# Autodesk Inventor assembly: Assy_linear_module
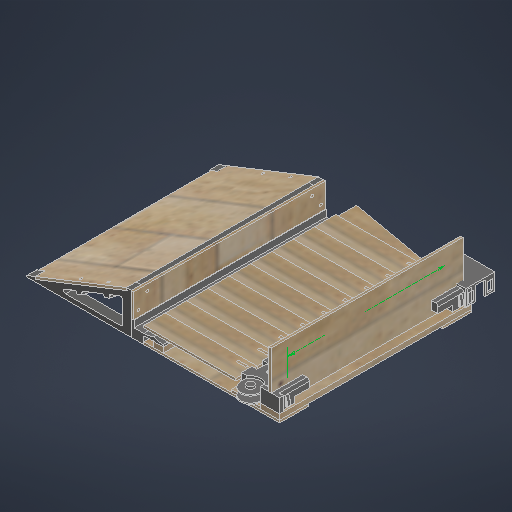
[picture p0: Inventor's stored thumbnail of the model, 512x512]
Saved by Autodesk Inventor 2026.3 (Build 303398000, 398)
## iProperties
Created: 2025-09-27
Part Number: Assy_linear_module
Document SubType Name: Assembly
Designer: hibik
Author: hibik
## Documents named in this file (15)
- D:\model\D2_Conveyor_2026\liniar_module\Assy_linear_module.iam
- D:\model\D2_Conveyor_2026\liniar_module\base.ipt
- D:\model\D2_Conveyor_2026\liniar_module\connector_base.ipt
- D:\model\D2_Conveyor_2026\liniar_module\back_upper.ipt
- D:\model\D2_Conveyor_2026\connectors\connector_male.ipt
- D:\model\D2_Conveyor_2026\liniar_module\belt_rail.ipt
- D:\model\D2_Conveyor_2026\liniar_module\front.ipt
- D:\model\D2_Conveyor_2026\belt\belt_linear.iam
- D:\model\D2_Conveyor_2026\liniar_module\front_rail.ipt
- D:\model\D2_Conveyor_2026\connectors\connetcor_female_cover.ipt
- D:\model\D2_Conveyor_2026\liniar_module\wall.ipt
- D:\model\D2_Conveyor_2026\liniar_module\Slope_Riner.ipt
- D:\model\D2_Conveyor_2026\liniar_module\Side_Wall_Riner.ipt
- D:\model\D2_Conveyor_2026\liniar_module\Spcer_Upper.ipt
- D:\model\D2_Conveyor_2026\liniar_module\Wall_Stand.ipt
## Components (17 placed, 14 different names)
1. base:1 — メイト:1, フラッシュ:1, フラッシュ:3, メイト:7, フラッシュ:7, フラッシュ:8, フラッシュ:9, メイト:12, フラッシュ:11
2. connector_base:1 — メイト:1, フラッシュ:1, フラッシュ:3, メイト:3, フラッシュ:5, フラッシュ:6, メイト:4, メイト:5, メイト:6, メイト:8, メイト:9, メイト:10, メイト:11, メイト:13, メイト:14, メイト:19
3. base:2 — メイト:3, フラッシュ:5, フラッシュ:6
4. connector_male:7 — メイト:9, メイト:10, メイト:11, メイト:16
5. connector_male:8 — メイト:4, メイト:5, メイト:6, メイト:17, メイト:18
6. belt_rail:1 — メイト:7, フラッシュ:7, メイト:8, 正接:1
7. front:1 — フラッシュ:8, フラッシュ:9, メイト:12, フラッシュ:12, フラッシュ:13, フラッシュ:14
8. back_upper:1 — フラッシュ:10, メイト:13, メイト:14, メイト:15
9. belt_linear:1 [sub-assembly] — メイト:15, 正接:1, フラッシュ:11
10. front_rail:1 — フラッシュ:12, フラッシュ:13, フラッシュ:14, フラッシュ:25, フラッシュ:26, メイト:24
11. connetcor_female_cover:1 — メイト:16
12. wall:1 — メイト:17, メイト:18, メイト:19
13. Slope_Riner:1 — メイト:20, メイト:21, フラッシュ:23, フラッシュ:24, メイト:22, メイト:23
14. Wall_Stand:2 — メイト:21, フラッシュ:23, メイト:23, フラッシュ:25, フラッシュ:26, メイト:24, 回転:1
15. Wall_Stand:3 — メイト:20, フラッシュ:24, メイト:22, メイト:25
16. Side_Wall_Riner:1 — メイト:25, 回転:1, メイト:26, 回転:2
17. Spcer_Upper:1 — メイト:26, 回転:2
## Relationships (44: Mate 25, Flush 16, RevoluteJoint 2, Tangent 1)
- メイト:1 [Mate]: base:1 ↔ connector_base:1
- フラッシュ:1 [Flush]: base:1 ↔ connector_base:1
- フラッシュ:3 [Flush]: base:1 ↔ connector_base:1
- メイト:3 [Mate]: connector_base:1 ↔ base:2
- フラッシュ:5 [Flush]: connector_base:1 ↔ base:2
- フラッシュ:6 [Flush]: connector_base:1 ↔ base:2
- メイト:4 [Mate]: connector_base:1 ↔ connector_male:8
- メイト:5 [Mate]: connector_base:1 ↔ connector_male:8
- メイト:6 [Mate]: connector_base:1 ↔ connector_male:8
- メイト:7 [Mate]: base:1 ↔ belt_rail:1
- フラッシュ:7 [Flush]: base:1 ↔ belt_rail:1
- メイト:8 [Mate]: connector_base:1 ↔ belt_rail:1
- メイト:9 [Mate]: connector_base:1 ↔ connector_male:7
- メイト:10 [Mate]: connector_base:1 ↔ connector_male:7
- メイト:11 [Mate]: connector_base:1 ↔ connector_male:7
- フラッシュ:8 [Flush]: base:1 ↔ front:1
- フラッシュ:9 [Flush]: base:1 ↔ front:1
- メイト:12 [Mate]: base:1 ↔ front:1
- フラッシュ:10 [Flush]: back_upper:1
- メイト:13 [Mate]: connector_base:1 ↔ back_upper:1
- メイト:14 [Mate]: connector_base:1 ↔ back_upper:1
- メイト:15 [Mate]: back_upper:1 ↔ belt_linear:1
- 正接:1 [Tangent]: belt_rail:1 ↔ belt_linear:1
- フラッシュ:11 [Flush]: base:1 ↔ belt_linear:1
- フラッシュ:12 [Flush]: front:1 ↔ front_rail:1
- フラッシュ:13 [Flush]: front:1 ↔ front_rail:1
- フラッシュ:14 [Flush]: front:1 ↔ front_rail:1
- メイト:16 [Mate]: connector_male:7 ↔ connetcor_female_cover:1
- メイト:17 [Mate]: connector_male:8 ↔ wall:1
- メイト:18 [Mate]: connector_male:8 ↔ wall:1
- メイト:19 [Mate]: connector_base:1 ↔ wall:1
- メイト:20 [Mate]: Slope_Riner:1 ↔ Wall_Stand:3
- メイト:21 [Mate]: Slope_Riner:1 ↔ Wall_Stand:2
- フラッシュ:23 [Flush]: Slope_Riner:1 ↔ Wall_Stand:2
- フラッシュ:24 [Flush]: Slope_Riner:1 ↔ Wall_Stand:3
- メイト:22 [Mate]: Slope_Riner:1 ↔ Wall_Stand:3
- メイト:23 [Mate]: Slope_Riner:1 ↔ Wall_Stand:2
- フラッシュ:25 [Flush]: front_rail:1 ↔ Wall_Stand:2
- フラッシュ:26 [Flush]: front_rail:1 ↔ Wall_Stand:2
- メイト:24 [Mate]: front_rail:1 ↔ Wall_Stand:2
- メイト:25 [Mate]: Wall_Stand:3 ↔ Side_Wall_Riner:1
- 回転:1 [RevoluteJoint]: Wall_Stand:2 ↔ Side_Wall_Riner:1
- メイト:26 [Mate]: Side_Wall_Riner:1 ↔ Spcer_Upper:1
- 回転:2 [RevoluteJoint]: Side_Wall_Riner:1 ↔ Spcer_Upper:1
